# Autodesk Inventor assembly: lifter_3
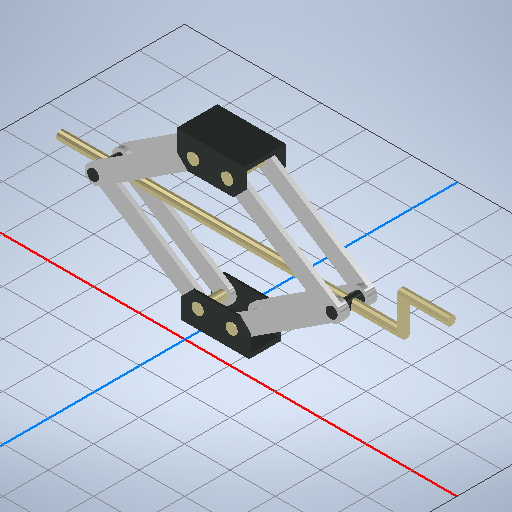
[picture p0: Inventor's stored thumbnail of the model, 512x512]
Saved by Autodesk Inventor 2025 (Build 290162000, 162)
## iProperties
Created: 2025-02-05
Part Number: lifter_3
Document SubType Name: Assembly
Designer: piotr
Author: piotr
## Documents named in this file (19)
- C:\Users\piotr\OneDrive\Pulpit\lifter_3\lifter_3.iam
- C:\Users\piotr\OneDrive\Pulpit\lifter_3\baza.ipt
- C:\Users\piotr\OneDrive\Pulpit\lifter_3\nitR1.ipt
- C:\Users\piotr\OneDrive\Pulpit\lifter_3\ramieR1.ipt
- C:\Users\piotr\OneDrive\Pulpit\lifter_3\ramieR2.ipt
- C:\Users\piotr\OneDrive\Pulpit\lifter_3\nitR2.ipt
- C:\Users\piotr\OneDrive\Pulpit\lifter_3\korona.ipt
- C:\Users\piotr\OneDrive\Pulpit\lifter_3\nitR3.ipt
- C:\Users\piotr\OneDrive\Pulpit\lifter_3\szynka.ipt
- C:\Users\piotr\OneDrive\Pulpit\lifter_3\ramieR1_MIR1.ipt
- C:\Users\piotr\OneDrive\Pulpit\lifter_3\ramieR2_MIR1.ipt
- C:\Users\piotr\OneDrive\Pulpit\lifter_3\nitR1_MIR.ipt
- C:\Users\piotr\OneDrive\Pulpit\lifter_3\ramieR1_MIR2.ipt
- C:\Users\piotr\OneDrive\Pulpit\lifter_3\ramieR2_MIR2.ipt
- C:\Users\piotr\OneDrive\Pulpit\lifter_3\nitR2_MIR.ipt
- C:\Users\piotr\OneDrive\Pulpit\lifter_3\nitR3_MIR.ipt
- C:\Users\piotr\OneDrive\Pulpit\lifter_3\ramieR1_MIR1_MIR.ipt
- C:\Users\piotr\OneDrive\Pulpit\lifter_3\ramieR2_MIR1_MIR.ipt
- C:\Users\piotr\OneDrive\Pulpit\lifter_3\korba.ipt
## Components (18 placed, 18 different names)
1. baza:1 — Mate:1, Angle:1, Flush:1, Flush:3, Flush:4, Flush:7, Insert:1, Insert:2, Flush:16, Flush:17, Mate:5, Flush:18, Flush:19, Insert:9, Insert:14, Insert:17, Mate:11
2. nitR1:1 — Flush:1, Flush:2, Insert:1
3. ramieR1:1 — Flush:3, Flush:4, Flush:5, Flush:6, Flush:7, Flush:8, Flush:9, Insert:2, Insert:3
4. ramieR2:1 — Flush:5, Flush:6, Flush:10, Flush:11, Insert:4, Mate:3
5. nitR2:1 — Flush:8, Flush:9, Insert:3, Insert:4, Insert:7, Insert:8, Flush:24, Mate:12, Tangent:1
6. korona:1 — Flush:10, Flush:11, Flush:12, Flush:13, Flush:14, Mate:2, Mate:3, Flush:15, Insert:5, Mate:4, Mate:5, Insert:6, Insert:15, Insert:16, Insert:18, Flush:28
7. nitR3:1 — Flush:12, Flush:13, Flush:14, Mate:2, Insert:5
8. szynka:1 — Flush:16, Flush:17, Mate:4
9. ramieR3:1 — Mate:6, Mate:7, Insert:8, Insert:9
10. ramieR4:1 — Mate:6, Mate:7, Insert:6, Insert:7
11. nitL1:1 — Mate:8, Insert:14
12. ramieL1:1 — Mate:9, Mate:10, Insert:10, Flush:20, Flush:21, Mate:11
13. ramieL2:1 — Mate:9, Mate:10, Insert:11, Insert:18
14. nitL2:1 — Insert:10, Insert:11, Flush:20, Flush:21, Insert:12, Insert:13, Mate:12, Tangent:2
15. nitL3:1 — Insert:15
16. ramieL3:1 — Insert:12, Flush:22, Flush:23, Insert:17
17. ramieL4:1 — Insert:13, Flush:22, Flush:23, Insert:16
18. korba:1 — Flush:25, Flush:26, Flush:27, Tangent:1, Tangent:2, Flush:28
## Relationships (61: Flush 28, Insert 18, Mate 12, Tangent 2, Angle 1)
- Mate:1: baza:1
- Angle:1 (0 deg): baza:1
- Flush:1: baza:1 ↔ nitR1:1
- Flush:2: nitR1:1
- Flush:3: baza:1 ↔ ramieR1:1
- Flush:4: baza:1 ↔ ramieR1:1
- Flush:5: ramieR1:1 ↔ ramieR2:1
- Flush:6: ramieR1:1 ↔ ramieR2:1
- Flush:7: baza:1 ↔ ramieR1:1
- Flush:8: ramieR1:1 ↔ nitR2:1
- Flush:9: ramieR1:1 ↔ nitR2:1
- Flush:10: ramieR2:1 ↔ korona:1
- Flush:11: ramieR2:1 ↔ korona:1
- Flush:12: korona:1 ↔ nitR3:1
- Flush:13: korona:1 ↔ nitR3:1
- Flush:14 (-37.5 mm): korona:1 ↔ nitR3:1
- Insert:1: baza:1 ↔ nitR1:1
- Insert:2: baza:1 ↔ ramieR1:1
- Insert:3: ramieR1:1 ↔ nitR2:1
- Insert:4: ramieR2:1 ↔ nitR2:1
- Mate:2: korona:1 ↔ nitR3:1
- Mate:3: ramieR2:1 ↔ korona:1
- Flush:15 (100 mm): korona:1
- Flush:16: baza:1 ↔ szynka:1
- Flush:17: baza:1 ↔ szynka:1
- Insert:5: korona:1 ↔ nitR3:1
- Mate:4: korona:1 ↔ szynka:1
- Mate:5 (160 mm): baza:1 ↔ korona:1
- Flush:18 (-35 mm): baza:1
- Flush:19 (-75 mm): baza:1
- Mate:6: ramieR3:1 ↔ ramieR4:1
- Mate:7: ramieR3:1 ↔ ramieR4:1
- Insert:6: korona:1 ↔ ramieR4:1
- Insert:7: nitR2:1 ↔ ramieR4:1
- Insert:8: nitR2:1 ↔ ramieR3:1
- Insert:9: baza:1 ↔ ramieR3:1
- Mate:8: nitL1:1
- Mate:9: ramieL1:1 ↔ ramieL2:1
- Mate:10: ramieL1:1 ↔ ramieL2:1
- Insert:10: ramieL1:1 ↔ nitL2:1
- Insert:11: ramieL2:1 ↔ nitL2:1
- Flush:20: ramieL1:1 ↔ nitL2:1
- Flush:21: ramieL1:1 ↔ nitL2:1
- Insert:12: nitL2:1 ↔ ramieL3:1
- Insert:13: nitL2:1 ↔ ramieL4:1
- Flush:22: ramieL3:1 ↔ ramieL4:1
- Flush:23: ramieL3:1 ↔ ramieL4:1
- Insert:14: baza:1 ↔ nitL1:1
- Insert:15: korona:1 ↔ nitL3:1
- Insert:16: korona:1 ↔ ramieL4:1
- Insert:17: baza:1 ↔ ramieL3:1
- Insert:18: korona:1 ↔ ramieL2:1
- Mate:11: baza:1 ↔ ramieL1:1
- Flush:24: nitR2:1
- Mate:12: nitR2:1 ↔ nitL2:1
- Flush:25: korba:1
- Flush:26: korba:1
- Flush:27: korba:1
- Tangent:1: nitR2:1 ↔ korba:1
- Tangent:2: nitL2:1 ↔ korba:1
- Flush:28 (300 mm): korona:1 ↔ korba:1
